# Autodesk Inventor assembly: ButtonAssembly
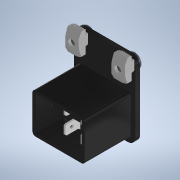
[picture p0: Inventor's stored thumbnail of the model, 180x180]
Saved by Autodesk Inventor 2020.2 (Build 242310000, 310)
## iProperties
Created: 2020-08-24
Part Number: ButtonAssembly
Document SubType Name: Assembly
Designer: JK
Author: JK
## Documents named in this file (5)
- C:\Users\JK\Documents\Inventor\Anet Upgrade\ButtonAssembly.iam
- C:\Users\JK\Documents\Inventor\Anet Upgrade\ButtonBox.ipt
- C:\Users\JK\Documents\Inventor\Anet Upgrade\RockerSwitch.ipt
- C:\Users\JK\Documents\Inventor\Anet Upgrade\M5x8BoltFlatHead.ipt
- C:\Users\JK\Documents\Inventor\Anet Upgrade\T_Slot_Nut_Dropin_3030m5ipt.ipt
## Components (6 placed, 4 different names)
1. ButtonBox:1 — Mate:1, Flush:1, Flush:2, Mate:2, Mate:3, Mate:4, Angle:1, Mate:7
2. RockerSwitch:1 — Mate:1, Flush:1, Flush:2
3. M5x8BoltFlatHead:1 — Mate:2, Mate:4, Flush:3, Mate:5
4. M5x8BoltFlatHead:2 — Mate:3, Flush:3, Mate:6
5. T_Slot_Nut_Dropin_3030m5ipt:1 — Mate:5, Flush:4, Angle:1, Mate:7
6. T_Slot_Nut_Dropin_3030m5ipt:2 — Mate:6, Flush:4
## Relationships (12: Mate 7, Flush 4, Angle 1)
- Mate:1: ButtonBox:1 ↔ RockerSwitch:1
- Flush:1 (2 mm): ButtonBox:1 ↔ RockerSwitch:1
- Flush:2 (5 mm): ButtonBox:1 ↔ RockerSwitch:1
- Mate:2: ButtonBox:1 ↔ M5x8BoltFlatHead:1
- Mate:3: ButtonBox:1 ↔ M5x8BoltFlatHead:2
- Mate:4: ButtonBox:1 ↔ M5x8BoltFlatHead:1
- Flush:3: M5x8BoltFlatHead:1 ↔ M5x8BoltFlatHead:2
- Mate:5: M5x8BoltFlatHead:1 ↔ T_Slot_Nut_Dropin_3030m5ipt:1
- Mate:6: M5x8BoltFlatHead:2 ↔ T_Slot_Nut_Dropin_3030m5ipt:2
- Flush:4: T_Slot_Nut_Dropin_3030m5ipt:1 ↔ T_Slot_Nut_Dropin_3030m5ipt:2
- Angle:1 (0 deg): ButtonBox:1 ↔ T_Slot_Nut_Dropin_3030m5ipt:1
- Mate:7: ButtonBox:1 ↔ T_Slot_Nut_Dropin_3030m5ipt:1
